# Autodesk Inventor assembly: Foot assembly
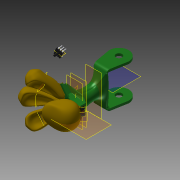
[picture p0: Inventor's stored thumbnail of the model, 180x180]
Saved by Autodesk Inventor 2015 (Build 190159000, 159)
## iProperties
Created: 2015-03-24
Part Number: Foot assembly
Document SubType Name: Assembly
Designer: Henke
Author: Henke
## Documents named in this file (5)
- D:\Study_and_Projects\KTH\KEX i robotik\CAD\Foot assembly.iam
- D:\Study_and_Projects\KTH\KEX i robotik\CAD\FootConnector.ipt
- D:\Study_and_Projects\KTH\KEX i robotik\CAD\Pressure sensor.ipt
- D:\Study_and_Projects\KTH\KEX i robotik\CAD\Foot Puff Big.ipt
- D:\Study_and_Projects\KTH\KEX i robotik\CAD\Foot Small Puff.ipt
## Components (6 placed, 4 different names)
1. FootConnector:1 — Mate:1, Mate:2, Mate:3, Mate:4, Mate:5, Mate:6, Mate:7, Mate:8, Mate:9, Mate:10, Mate:11, Mate:12
2. Pressure sensor:1
3. Foot Puff Big:1 — Mate:1, Mate:2, Mate:3
4. Foot Small Puff:1 — Mate:4, Mate:5, Mate:6
5. Foot Small Puff:2 — Mate:7, Mate:8, Mate:9
6. Foot Small Puff:3 — Mate:10, Mate:11, Mate:12
## Relationships (12: Mate 12)
- Mate:1: FootConnector:1 ↔ Foot Puff Big:1
- Mate:2: FootConnector:1 ↔ Foot Puff Big:1
- Mate:3: FootConnector:1 ↔ Foot Puff Big:1
- Mate:4: FootConnector:1 ↔ Foot Small Puff:1
- Mate:5: FootConnector:1 ↔ Foot Small Puff:1
- Mate:6: FootConnector:1 ↔ Foot Small Puff:1
- Mate:7: FootConnector:1 ↔ Foot Small Puff:2
- Mate:8: FootConnector:1 ↔ Foot Small Puff:2
- Mate:9: FootConnector:1 ↔ Foot Small Puff:2
- Mate:10: FootConnector:1 ↔ Foot Small Puff:3
- Mate:11: FootConnector:1 ↔ Foot Small Puff:3
- Mate:12: FootConnector:1 ↔ Foot Small Puff:3
